# Autodesk Inventor assembly: EnsambleGarraSTD
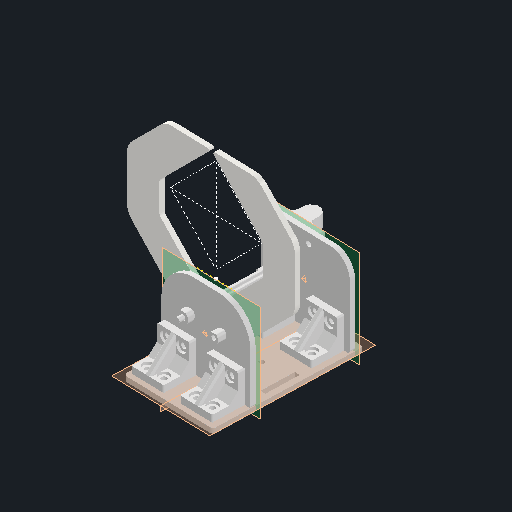
[picture p0: Inventor's stored thumbnail of the model, 512x512]
Saved by Autodesk Inventor 2026.3 (Build 303398000, 398)
## iProperties
Created: 2026-04-16
Part Number: EnsambleGarraSTD
Document SubType Name: Assembly
Designer: Jose Carlos
Author: Jose Carlos
## Documents named in this file (16)
- C:\Users\Caro\JoseCarlos\TEC\TFG\Inventor\PiezasSTD\EnsambleGarraSTD.iam
- C:\Users\Caro\JoseCarlos\TEC\TFG\Inventor\PiezasSTD\PlacaFrontalSTD.ipt
- C:\Users\Caro\JoseCarlos\TEC\TFG\Inventor\PiezasSTD\T.ipt
- C:\Users\Caro\JoseCarlos\TEC\TFG\Inventor\PiezasSTD\PlacaBaseGarraSTD.ipt
- C:\Users\Caro\JoseCarlos\TEC\TFG\Inventor\PiezasSTD\BaseEngranes.ipt
- C:\Users\Caro\JoseCarlos\TEC\TFG\Inventor\PiezasSTD\EnsambleGarraSTD\Design Accelerator\Engranajes rectos2.iam
- C:\Users\Caro\JoseCarlos\TEC\TFG\Inventor\PiezasSTD\PlacaBaseGarraPotenciaSTD.ipt
- C:\Users\Caro\JoseCarlos\TEC\TFG\Inventor\PiezasSTD\EjecilindroGarraSTD.ipt
- C:\Users\Caro\JoseCarlos\TEC\TFG\Inventor\PiezasSTD\BaseEjeConicos.ipt
- C:\Users\Caro\JoseCarlos\TEC\TFG\Inventor\PiezasSTD\EnsambleGarraSTD\Design Accelerator\Engranajes biselados1.iam
- C:\Users\Caro\JoseCarlos\TEC\TFG\Inventor\PiezasSTD\EjeCilintroSuperiorGarra.ipt
- C:\Users\Caro\JoseCarlos\TEC\TFG\Inventor\PiezasSTD\SoporteEjes.ipt
- C:\Users\Caro\JoseCarlos\TEC\TFG\Inventor\PiezasSTD\Acoplador.ipt
- C:\Users\Caro\JoseCarlos\TEC\TFG\Inventor\PiezasSTD\TapónEje.ipt
- C:\Users\Caro\JoseCarlos\TEC\TFG\Inventor\PiezasSTD\ReyenedorTornillo3M.ipt
- C:\Users\Caro\JoseCarlos\TEC\TFG\Inventor\PiezasSTD\RetenedorEjeGarraVerticalSuperior.ipt
## Components (18 placed, 15 different names)
1. PlacaFrontalSTD:1 — Coincidencia:1, Coincidencia:2, Coincidencia:3, Coincidencia:4, Nivelación:1, Coincidencia:5, Coincidencia:6, Coincidencia:9, Coincidencia:10, Coincidencia:11, Coincidencia:12, Coincidencia:13, Coincidencia:14, Coincidencia:16, Coincidencia:17, Nivelación:6, Nivelación:7
2. T:1 — Coincidencia:1, Coincidencia:2
3. T:2 — Coincidencia:3, Coincidencia:4
4. PlacaBaseGarraSTD:1 — Nivelación:1, Coincidencia:5, Coincidencia:6, Nivelación:2, Nivelación:3, Coincidencia:18, Nivelación:14, Nivelación:15, Coincidencia:21
5. BaseEngranes:1 — Nivelación:2, Nivelación:3, Coincidencia:7, Coincidencia:8
6. Engranajes rectos:1 [sub-assembly] — Coincidencia:7, Coincidencia:8, Coincidencia:18, Nivelación:17, Nivelación:18, Nivelación:19
7. T:3 — Coincidencia:9, Coincidencia:10, Coincidencia:11
8. T:4 — Coincidencia:12, Coincidencia:13, Coincidencia:14, Coincidencia:15
9. PlacaBaseGarraPotenciaSTD:1 — Coincidencia:15, Coincidencia:16, Coincidencia:17, Nivelación:8
10. EjecilindroGarraSTD:1 — Nivelación:16, Coincidencia:21, Nivelación:17
11. BaseEjeConicos:1 — Nivelación:6, Nivelación:7, Nivelación:8, Coincidencia:19, Coincidencia:20
12. Engranajes biselados:1 [sub-assembly] — Coincidencia:19, Coincidencia:20, Nivelación:9, Nivelación:16, Nivelación:21
13. EjeCilintroSuperiorGarra:1 — Nivelación:9, Nivelación:10, Nivelación:11, Nivelación:20, Nivelación:21
14. SoporteEjes:1 — Nivelación:10
15. Acoplador:1 — Nivelación:11, Nivelación:20
16. TapónEje:1
17. ReyenedorTornillo3M:1 — Nivelación:14, Nivelación:15
18. RetenedorEjeGarraVerticalSuperior:1 — Nivelación:18, Nivelación:19
## Relationships (38: Mate 21, Flush 17)
- Coincidencia:1 [Mate]: PlacaFrontalSTD:1 ↔ T:1
- Coincidencia:2 [Mate]: PlacaFrontalSTD:1 ↔ T:1
- Coincidencia:3 [Mate]: PlacaFrontalSTD:1 ↔ T:2
- Coincidencia:4 [Mate]: PlacaFrontalSTD:1 ↔ T:2
- Nivelación:1 [Flush]: PlacaFrontalSTD:1 ↔ PlacaBaseGarraSTD:1
- Coincidencia:5 [Mate]: PlacaFrontalSTD:1 ↔ PlacaBaseGarraSTD:1
- Coincidencia:6 [Mate]: PlacaFrontalSTD:1 ↔ PlacaBaseGarraSTD:1
- Nivelación:2 [Flush]: PlacaBaseGarraSTD:1 ↔ BaseEngranes:1
- Nivelación:3 [Flush]: PlacaBaseGarraSTD:1 ↔ BaseEngranes:1
- Coincidencia:7 [Mate]: BaseEngranes:1 ↔ Engranajes rectos:1
- Coincidencia:8 [Mate]: BaseEngranes:1 ↔ Engranajes rectos:1
- Coincidencia:9 [Mate]: PlacaFrontalSTD:1 ↔ T:3
- Coincidencia:10 [Mate]: PlacaFrontalSTD:1 ↔ T:3
- Coincidencia:11 [Mate]: PlacaFrontalSTD:1 ↔ T:3
- Coincidencia:12 [Mate]: PlacaFrontalSTD:1 ↔ T:4
- Coincidencia:13 [Mate]: PlacaFrontalSTD:1 ↔ T:4
- Coincidencia:14 [Mate]: PlacaFrontalSTD:1 ↔ T:4
- Coincidencia:15 [Mate]: T:4 ↔ PlacaBaseGarraPotenciaSTD:1
- Coincidencia:16 [Mate]: PlacaFrontalSTD:1 ↔ PlacaBaseGarraPotenciaSTD:1
- Coincidencia:17 [Mate]: PlacaFrontalSTD:1 ↔ PlacaBaseGarraPotenciaSTD:1
- Coincidencia:18 [Mate]: PlacaBaseGarraSTD:1 ↔ Engranajes rectos:1
- Nivelación:6 [Flush]: PlacaFrontalSTD:1 ↔ BaseEjeConicos:1
- Nivelación:7 [Flush]: PlacaFrontalSTD:1 ↔ BaseEjeConicos:1
- Nivelación:8 [Flush]: PlacaBaseGarraPotenciaSTD:1 ↔ BaseEjeConicos:1
- Coincidencia:19 [Mate]: BaseEjeConicos:1 ↔ Engranajes biselados:1
- Coincidencia:20 [Mate]: BaseEjeConicos:1 ↔ Engranajes biselados:1
- Nivelación:9 [Flush]: Engranajes biselados:1 ↔ EjeCilintroSuperiorGarra:1
- Nivelación:10 [Flush]: EjeCilintroSuperiorGarra:1 ↔ SoporteEjes:1
- Nivelación:11 [Flush]: EjeCilintroSuperiorGarra:1 ↔ Acoplador:1
- Nivelación:14 [Flush]: PlacaBaseGarraSTD:1 ↔ ReyenedorTornillo3M:1
- Nivelación:15 [Flush]: PlacaBaseGarraSTD:1 ↔ ReyenedorTornillo3M:1
- Nivelación:16 [Flush]: EjecilindroGarraSTD:1 ↔ Engranajes biselados:1
- Coincidencia:21 [Mate]: PlacaBaseGarraSTD:1 ↔ EjecilindroGarraSTD:1
- Nivelación:17 [Flush] (0.2 mm): Engranajes rectos:1 ↔ EjecilindroGarraSTD:1
- Nivelación:18 [Flush]: Engranajes rectos:1 ↔ RetenedorEjeGarraVerticalSuperior:1
- Nivelación:19 [Flush]: Engranajes rectos:1 ↔ RetenedorEjeGarraVerticalSuperior:1
- Nivelación:20 [Flush]: EjeCilintroSuperiorGarra:1 ↔ Acoplador:1
- Nivelación:21 [Flush]: Engranajes biselados:1 ↔ EjeCilintroSuperiorGarra:1
